# Autodesk Inventor assembly: Metal_Light_Housing
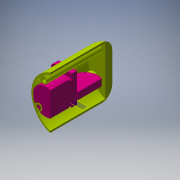
[picture p0: Inventor's stored thumbnail of the model, 180x180]
Saved by Autodesk Inventor 2016 (Build 200138000, 138)
## iProperties
Created: 2017-12-20
Part Number: Metal_Light_Housing
Document SubType Name: Assembly
Designer: Student
Author: Student
## Documents named in this file (3)
- C:\Users\Student\Documents\CAD\Bike Light Housing\Metal_Light_Housing.iam
- C:\Users\Student\Documents\CAD\Bike Light Housing\Light Circuit.ipt
- C:\Users\Student\Documents\CAD\Bike Light Housing\MetalFrame.ipt
## Components (2 placed, 2 different names)
1. Light Circuit:1
2. MetalFrame:1 — Angle:1
## Relationships (1: Angle 1)
- Angle:1 (0 deg): MetalFrame:1
